# Autodesk Inventor assembly: Motor_MIR
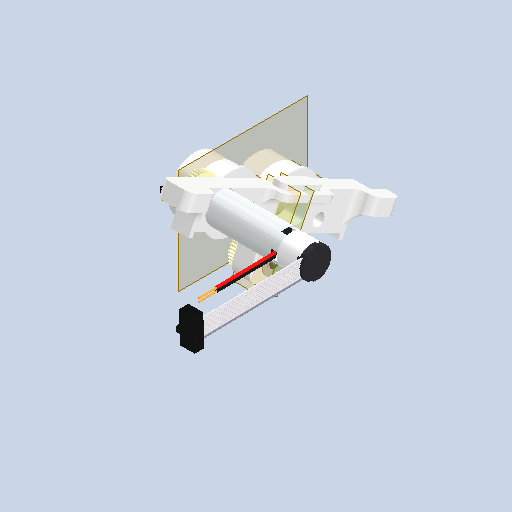
[picture p0: Inventor's stored thumbnail of the model, 512x512]
Saved by Autodesk Inventor 2022 (Build 260153000, 153)
## iProperties
Created: 2021-09-24
Part Number: Motor_MIR
Document SubType Name: Assembly
Designer: shiokaze
Mass: 31.1386 g
Surface Area: 214.594 cm^2
Volume: 14.9157 cm^3
Author: shiok
## Documents named in this file (8)
- C:\Users\Yazawa\Documents\GitHub\murakumo\inventor\Motor_MIR.iam
- C:\Users\Yazawa\Documents\GitHub\murakumo\inventor\Tire_MIR2.iam
- C:\Users\Yazawa\Documents\GitHub\murakumo\inventor\MotorBracketv2_MIR.ipt
- C:\Users\Yazawa\Documents\GitHub\murakumo\inventor\maxon DCX 10L_MIR2.iam
- C:\Users\Yazawa\Documents\GitHub\murakumo\inventor\FL674ZZ_MIR_MIR.ipt
- C:\Users\Yazawa\Documents\GitHub\murakumo\inventor\piniongear_41_middle_MIR2.ipt
- C:\Users\Yazawa\Documents\GitHub\murakumo\inventor\piniongear_41_src_MIR2.ipt
- C:\Users\Yazawa\Documents\GitHub\murakumo\inventor\shaft_short_MIR2.ipt
## Components (9 placed, 7 different names)
1. Tire_MIR2:1 [sub-assembly] — メイト:11, メイト:6, フラッシュ:1, 対称度:1
2. MotorBracketv2_MIR:1 — メイト:11, メイト:6, メイト:7, メイト:10, メイト:8, メイト:4, メイト:3, メイト:2, メイト:1
3. Tire_MIR2:2 [sub-assembly] — フラッシュ:1, メイト:7, フラッシュ:2, フラッシュ:3, 対称度:1
4. maxon DCX 10L_MIR2:1 [sub-assembly] — メイト:10, メイト:8, メイト:9
5. FL674ZZ_MIR_MIR:1 — メイト:4, メイト:3
6. FL674ZZ_MIR_MIR:2 — メイト:2, メイト:1, メイト:5
7. piniongear_41_middle_MIR2:1 — フラッシュ:2, 挿入:6
8. piniongear_41_src_MIR2:1 — メイト:9, フラッシュ:3
9. shaft_short_MIR2:1 — メイト:5, 挿入:6
## Relationships (16: Mate 11, Flush 3, Insert 1, Symmetry 1)
- メイト:11 [Mate] (1 mm): Tire_MIR2:1 ↔ MotorBracketv2_MIR:1
- メイト:6 [Mate]: Tire_MIR2:1 ↔ MotorBracketv2_MIR:1
- フラッシュ:1 [Flush]: Tire_MIR2:1 ↔ Tire_MIR2:2
- メイト:7 [Mate]: MotorBracketv2_MIR:1 ↔ Tire_MIR2:2
- メイト:10 [Mate]: MotorBracketv2_MIR:1 ↔ maxon DCX 10L_MIR2:1
- メイト:8 [Mate]: MotorBracketv2_MIR:1 ↔ maxon DCX 10L_MIR2:1
- メイト:4 [Mate]: MotorBracketv2_MIR:1 ↔ FL674ZZ_MIR_MIR:1
- メイト:3 [Mate]: MotorBracketv2_MIR:1 ↔ FL674ZZ_MIR_MIR:1
- メイト:2 [Mate]: MotorBracketv2_MIR:1 ↔ FL674ZZ_MIR_MIR:2
- メイト:1 [Mate]: MotorBracketv2_MIR:1 ↔ FL674ZZ_MIR_MIR:2
- フラッシュ:2 [Flush]: Tire_MIR2:2 ↔ piniongear_41_middle_MIR2:1
- メイト:9 [Mate]: maxon DCX 10L_MIR2:1 ↔ piniongear_41_src_MIR2:1
- フラッシュ:3 [Flush]: Tire_MIR2:2 ↔ piniongear_41_src_MIR2:1
- メイト:5 [Mate]: FL674ZZ_MIR_MIR:2 ↔ shaft_short_MIR2:1
- 挿入:6 [Insert]: piniongear_41_middle_MIR2:1 ↔ shaft_short_MIR2:1
- 対称度:1 [Symmetry]: Tire_MIR2:1 ↔ Tire_MIR2:2
